# Autodesk Inventor assembly: bed_assembly
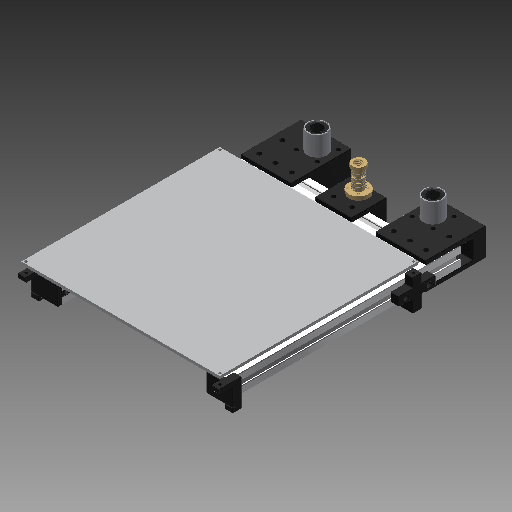
[picture p0: Inventor's stored thumbnail of the model, 512x512]
Saved by Autodesk Inventor 2018 (Build 220112000, 112)
## iProperties
Created: 2018-05-24
Part Number: bed_assembly
Document SubType Name: Assembly
Designer: Z. Deniz
Author: Z. Deniz
## Documents named in this file (13)
- C:\Users\zdeni\Desktop\3d\Yeni klasör\bed_assembly.iam
- C:\Users\zdeni\Desktop\3d\Yeni klasör\2020 Extrusion 160mm.ipt
- C:\Users\zdeni\Desktop\3d\Yeni klasör\2020 Extrusion 250mm.ipt
- C:\Users\zdeni\Desktop\3d\Yeni klasör\bed_pulley_holder.ipt
- C:\Users\zdeni\Desktop\3d\Yeni klasör\90 angle.ipt
- C:\Users\zdeni\Desktop\3d\Yeni klasör\HEATBED MK3.ipt
- C:\Users\zdeni\Desktop\3d\Yeni klasör\123LMK12LUU.ipt
- C:\Users\zdeni\Desktop\3d\Yeni klasör\bed_front_cover.ipt
- C:\Users\zdeni\Desktop\3d\Yeni klasör\bed_spring_holder_back.ipt
- C:\Users\zdeni\Desktop\3d\Yeni klasör\bed_spring_holder_front.ipt
- C:\Users\zdeni\Desktop\3d\Yeni klasör\bed_spring_holder_back_v2.ipt
- C:\Users\zdeni\Desktop\3d\Yeni klasör\z_nut_holder.ipt
- C:\Users\zdeni\Desktop\3d\Yeni klasör\123TR8_8(P4) Antibacklash Nut w. spring.ipt
## Components (20 placed, 12 different names)
1. 2020 Extrusion 160mm:1 — Mate:1, Flush:1, Flush:2, Flush:3, Mate:2, Flush:4, Mate:3, Mate:6, Mate:8, Mate:9, Mate:11, Mate:30, Mate:31
2. 2020 Extrusion 250mm:1 — Flush:3, Mate:2, Flush:4, Mate:4, Flush:5, Mate:7, Mate:18, Flush:7, Flush:8, Mate:24, Mate:25
3. bed_pulley_holder:1 — Mate:7, Mate:8, Mate:9, Tangent:2, Mate:17, Tangent:7, Mate:32
4. 2020 Extrusion 250mm:2 — Mate:1, Flush:1, Flush:2, Mate:5, Flush:6, Mate:10, Mate:12, Flush:9, Mate:19, Flush:10, Mate:27, Mate:28
5. 90 angle:1 — Mate:5, Mate:6, Flush:6
6. 90 angle:2 — Mate:3, Mate:4, Flush:5
7. bed_pulley_holder:2 — Mate:10, Mate:11, Mate:12, Mate:13, Tangent:1, Mate:16, Tangent:6
8. HEATBED MK3:1 — Flush:11, Tangent:3, Tangent:4, Mate:26, Tangent:5
9. 123LMK12LUU:1 — Tangent:1, Mate:16, Tangent:6
10. 123LMK12LUU:2 — Tangent:2, Mate:17, Tangent:7
11. bed_front_cover:1 — Mate:18, Flush:7, Flush:8, Mate:22, Flush:13, Mate:29
12. bed_front_cover:2 — Flush:9, Mate:19, Flush:10, Flush:11, Mate:20, Mate:21, Flush:12
13. bed_spring_holder_back:1
14. bed_spring_holder_front:1 — Mate:22, Flush:13, Tangent:3, Mate:26, Mate:29
15. bed_spring_holder_back:2
16. bed_spring_holder_front:2 — Mate:20, Mate:21, Flush:12
17. bed_spring_holder_back_v2:1 — Mate:24, Mate:25, Tangent:4
18. bed_spring_holder_back_v2:2 — Mate:27, Mate:28, Tangent:5
19. z_nut_holder:1 — Mate:30, Mate:31, Mate:32, Mate:33, Mate:34, Mate:35
20. 123TR8_8(P4) Antibacklash Nut w. spring:1 — Mate:33, Mate:34, Mate:35
## Relationships (52: Mate 32, Flush 13, Tangent 7)
- Mate:1: 2020 Extrusion 160mm:1 ↔ 2020 Extrusion 250mm:2
- Flush:1: 2020 Extrusion 160mm:1 ↔ 2020 Extrusion 250mm:2
- Flush:2 (17.5 mm): 2020 Extrusion 160mm:1 ↔ 2020 Extrusion 250mm:2
- Flush:3: 2020 Extrusion 160mm:1 ↔ 2020 Extrusion 250mm:1
- Mate:2: 2020 Extrusion 160mm:1 ↔ 2020 Extrusion 250mm:1
- Flush:4 (17.5 mm): 2020 Extrusion 160mm:1 ↔ 2020 Extrusion 250mm:1
- Mate:3: 2020 Extrusion 160mm:1 ↔ 90 angle:2
- Mate:4: 2020 Extrusion 250mm:1 ↔ 90 angle:2
- Flush:5 (1.5 mm): 2020 Extrusion 250mm:1 ↔ 90 angle:2
- Mate:5: 2020 Extrusion 250mm:2 ↔ 90 angle:1
- Mate:6: 2020 Extrusion 160mm:1 ↔ 90 angle:1
- Flush:6 (1.5 mm): 2020 Extrusion 250mm:2 ↔ 90 angle:1
- Mate:7: 2020 Extrusion 250mm:1 ↔ bed_pulley_holder:1
- Mate:8: 2020 Extrusion 160mm:1 ↔ bed_pulley_holder:1
- Mate:9: 2020 Extrusion 160mm:1 ↔ bed_pulley_holder:1
- Mate:10: 2020 Extrusion 250mm:2 ↔ bed_pulley_holder:2
- Mate:11: 2020 Extrusion 160mm:1 ↔ bed_pulley_holder:2
- Mate:12: 2020 Extrusion 250mm:2 ↔ bed_pulley_holder:2
- Mate:13: bed_pulley_holder:2
- Tangent:1: bed_pulley_holder:2 ↔ 123LMK12LUU:1
- Mate:16: bed_pulley_holder:2 ↔ 123LMK12LUU:1
- Tangent:2: bed_pulley_holder:1 ↔ 123LMK12LUU:2
- Mate:17: bed_pulley_holder:1 ↔ 123LMK12LUU:2
- Mate:18: 2020 Extrusion 250mm:1 ↔ bed_front_cover:1
- Flush:7: 2020 Extrusion 250mm:1 ↔ bed_front_cover:1
- Flush:8: 2020 Extrusion 250mm:1 ↔ bed_front_cover:1
- Flush:9: 2020 Extrusion 250mm:2 ↔ bed_front_cover:2
- Mate:19: 2020 Extrusion 250mm:2 ↔ bed_front_cover:2
- Flush:10: 2020 Extrusion 250mm:2 ↔ bed_front_cover:2
- Flush:11 (2 mm): HEATBED MK3:1 ↔ bed_front_cover:2
- Mate:20: bed_front_cover:2 ↔ bed_spring_holder_front:2
- Mate:21: bed_front_cover:2 ↔ bed_spring_holder_front:2
- Flush:12: bed_front_cover:2 ↔ bed_spring_holder_front:2
- Mate:22: bed_front_cover:1 ↔ bed_spring_holder_front:1
- Flush:13: bed_front_cover:1 ↔ bed_spring_holder_front:1
- Tangent:3: HEATBED MK3:1 ↔ bed_spring_holder_front:1
- Mate:24: 2020 Extrusion 250mm:1 ↔ bed_spring_holder_back_v2:1
- Mate:25: 2020 Extrusion 250mm:1 ↔ bed_spring_holder_back_v2:1
- Tangent:4: HEATBED MK3:1 ↔ bed_spring_holder_back_v2:1
- Mate:26 (7.5 mm): HEATBED MK3:1 ↔ bed_spring_holder_front:1
- Mate:27: 2020 Extrusion 250mm:2 ↔ bed_spring_holder_back_v2:2
- Mate:28: 2020 Extrusion 250mm:2 ↔ bed_spring_holder_back_v2:2
- Tangent:5: HEATBED MK3:1 ↔ bed_spring_holder_back_v2:2
- Mate:29: bed_front_cover:1 ↔ bed_spring_holder_front:1
- Tangent:6: bed_pulley_holder:2 ↔ 123LMK12LUU:1
- Tangent:7: bed_pulley_holder:1 ↔ 123LMK12LUU:2
- Mate:30: 2020 Extrusion 160mm:1 ↔ z_nut_holder:1
- Mate:31: 2020 Extrusion 160mm:1 ↔ z_nut_holder:1
- Mate:32 (25 mm): bed_pulley_holder:1 ↔ z_nut_holder:1
- Mate:33: z_nut_holder:1 ↔ 123TR8_8(P4) Antibacklash Nut w. spring:1
- Mate:34: z_nut_holder:1 ↔ 123TR8_8(P4) Antibacklash Nut w. spring:1
- Mate:35: z_nut_holder:1 ↔ 123TR8_8(P4) Antibacklash Nut w. spring:1
## Named parameters: back_space = 17.5 mm
